# Autodesk Inventor assembly: Main Body
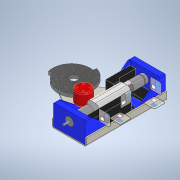
[picture p0: Inventor's stored thumbnail of the model, 180x180]
Saved by Autodesk Inventor 2022 (Build 260153000, 153)
## iProperties
Created: 2022-08-09
Part Number: Main Body
Document SubType Name: Assembly
Designer: Nick
Mass: 1403.94 g
Surface Area: 2459.61 cm^2
Volume: 453.242 cm^3
Density: 3.09755 g/cm^3
Author: Nick
## Documents named in this file (10)
- Y:\Projects\BattleBot\Main Body.iam
- Y:\Projects\BattleBot\Battery.ipt
- Y:\Projects\BattleBot\ESC.ipt
- Y:\Projects\BattleBot\Motor.ipt
- Y:\Projects\BattleBot\RC Reciever.ipt
- Y:\Projects\BattleBot\Base Plate.ipt
- Y:\Projects\BattleBot\Weapon.ipt
- Y:\Projects\BattleBot\Unmodified Motor.ipt
- Y:\Projects\BattleBot\Brushed ESC.ipt
- Y:\Projects\BattleBot\Motor Mount.ipt
## Components (13 placed, 9 different names)
1. Battery:1 — Mate:44, Mate:65, Mate:66
2. ESC:1 — Mate:45, Mate:46, Mate:47, Mate:66
3. RC Reciever:1 — Mate:53, Mate:62, Mate:64
4. Base Plate:1 — Mate:40, Flush:14, Flush:16, Mate:42, Mate:60, Mate:67
5. Weapon:1 — Insert:3
6. Unmodified Motor:1 — Mate:61
7. Motor:2 — Insert:1, Mate:65
8. Motor:3 — Insert:2
9. Brushed ESC:1 — Mate:50, Mate:51
10. Brushed ESC:2 — Mate:55, Mate:56, Mate:63
11. Motor Mount:1 — Insert:1, Mate:40, Flush:14, Mate:44, Mate:45, Mate:46, Mate:47, Mate:50, Mate:51, Mate:58, Flush:17, Mate:59, Mate:60
12. Motor Mount:2 — Insert:2, Flush:16, Mate:42, Mate:53, Mate:55, Mate:56, Mate:62, Mate:63, Mate:64, Mate:67
13. Base Plate:2 — Mate:58, Flush:17, Mate:59, Mate:61, Insert:3
## Relationships (27: Mate 21, Insert 3, Flush 3)
- Insert:1: Motor:2 ↔ Motor Mount:1
- Mate:40: Base Plate:1 ↔ Motor Mount:1
- Flush:14: Base Plate:1 ↔ Motor Mount:1
- Insert:2: Motor:3 ↔ Motor Mount:2
- Flush:16: Base Plate:1 ↔ Motor Mount:2
- Mate:42: Base Plate:1 ↔ Motor Mount:2
- Mate:44: Battery:1 ↔ Motor Mount:1
- Mate:45: ESC:1 ↔ Motor Mount:1
- Mate:46: ESC:1 ↔ Motor Mount:1
- Mate:47 (5 mm): ESC:1 ↔ Motor Mount:1
- Mate:50: Brushed ESC:1 ↔ Motor Mount:1
- Mate:51: Brushed ESC:1 ↔ Motor Mount:1
- Mate:53: RC Reciever:1 ↔ Motor Mount:2
- Mate:55: Brushed ESC:2 ↔ Motor Mount:2
- Mate:56: Brushed ESC:2 ↔ Motor Mount:2
- Mate:58: Motor Mount:1 ↔ Base Plate:2
- Flush:17: Motor Mount:1 ↔ Base Plate:2
- Mate:59: Motor Mount:1 ↔ Base Plate:2
- Mate:60: Base Plate:1 ↔ Motor Mount:1
- Mate:61: Unmodified Motor:1 ↔ Base Plate:2
- Insert:3 (16.825 mm): Weapon:1 ↔ Base Plate:2
- Mate:62: RC Reciever:1 ↔ Motor Mount:2
- Mate:63 (5 mm): Brushed ESC:2 ↔ Motor Mount:2
- Mate:64: RC Reciever:1 ↔ Motor Mount:2
- Mate:65 (6 mm): Battery:1 ↔ Motor:2
- Mate:66 (3 mm): Battery:1 ↔ ESC:1
- Mate:67: Base Plate:1 ↔ Motor Mount:2
